(part 1 of 2)
# Autodesk Inventor assembly: woodhouseV1
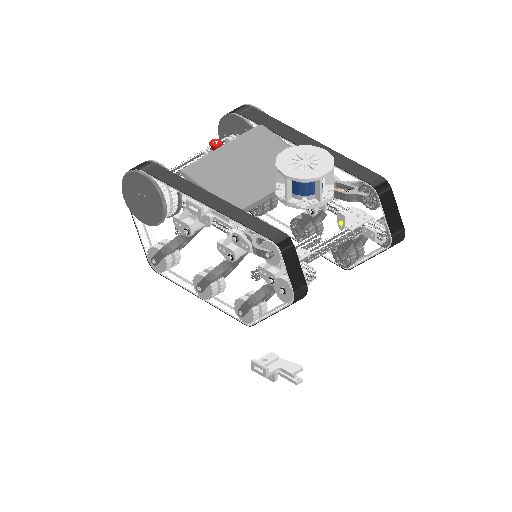
[picture p0: Inventor's stored thumbnail of the model, 512x512]
Saved by Autodesk Inventor 2025 (Build 290162000, 162)
## iProperties
Created: 2024-10-22
Part Number: woodhouseV1
Document SubType Name: Assembly
Designer: derm
Author: derm
## Documents named in this file (47)
- C:\Users\derm\Desktop\puppycat\woodhouseV1.iam
- C:\Users\derm\Desktop\puppycat\100MMshockUpper.ipt
- C:\Users\derm\Desktop\puppycat\100MMshockLower.ipt
- C:\Users\derm\Desktop\puppycat\swingarmBaseV2.ipt
- C:\Users\derm\Desktop\puppycat\6082rsBearing.ipt
- C:\Users\derm\Desktop\puppycat\92981A203_Alloy Steel Shoulder Screws\92981A203_Alloy Steel Shoulder Screws.ipt
- C:\Users\derm\Desktop\puppycat\swingarmV2.ipt
- C:\Users\derm\Desktop\puppycat\am-3298a 20 tooth Molded Tank Pulley Half Rev4\am-3298a 20 tooth Molded Tank Pulley Half Rev4.ipt
- C:\Users\derm\Desktop\puppycat\am3298_bearing_adapter.ipt
- C:\Users\derm\Desktop\puppycat\90237A130_High-Strength Steel Nylon-Insert Locknuts\90237A130_High-Strength Steel Nylon-Insert Locknuts.ipt
- C:\Users\derm\Desktop\puppycat\trackBase.ipt
- C:\Users\derm\Desktop\puppycat\moteur hoverboard\hoverboard_motor_assembly\hoverboard_motor_assembly.ipt
- C:\Users\derm\Desktop\puppycat\hoverboardPulleyAdapter.ipt
- C:\Users\derm\Desktop\puppycat\hoverboardMotorMount.ipt
- C:\Users\derm\Desktop\puppycat\idlerBaseV1.ipt
- C:\Users\derm\Desktop\puppycat\printedWheel.ipt
- C:\Users\derm\Desktop\puppycat\9002T445_Corrosion-Resistant Precision Compression Springs\9002T445_Corrosion-Resistant Precision Compression Springs.ipt
- C:\Users\derm\Desktop\puppycat\idlerV1.ipt
- C:\Users\derm\Desktop\puppycat\beltV2.ipt
- C:\Users\derm\Desktop\puppycat\springSpacerV1.ipt
- C:\Users\derm\Desktop\puppycat\swingarmBaseV4.ipt
- C:\Users\derm\Desktop\puppycat\swingarmBaseV4_mirror.ipt
- C:\Users\derm\Desktop\puppycat\swingarmV2_mirrored.ipt
- C:\Users\derm\Desktop\puppycat\91290A461_Alloy Steel Socket Head Screw\91290A461_Alloy Steel Socket Head Screw.ipt
- C:\Users\derm\Desktop\puppycat\94645A210_High-Strength Steel Nylon-Insert Locknut\94645A210_High-Strength Steel Nylon-Insert Locknut.ipt
- C:\Users\derm\Desktop\puppycat\91290A270_Alloy Steel Socket Head Screw\91290A270_Alloy Steel Socket Head Screw.ipt
- C:\Users\derm\Desktop\puppycat\horizontalStrut.ipt
- C:\Users\derm\Desktop\puppycat\4844N132_T-Slotted Framing Structural Bracket\4844N132_T-Slotted Framing Structural Bracket.ipt
- C:\Users\derm\Desktop\puppycat\4844N105_T-Slotted Framing Structural Bracket\4844N105_T-Slotted Framing Structural Bracket.ipt
- C:\Users\derm\Desktop\puppycat\lidarFOV.ipt
- C:\Users\derm\Desktop\puppycat\Motor driver ODRIVE V3.6\Motor driver ODRIVE V3.6.ipt
- C:\Users\derm\Desktop\puppycat\Zippy5000.ipt
- C:\Users\derm\Desktop\puppycat\50W 2Ohm Power Resistor\50W 2Ohm Power Resistor.ipt
- C:\Users\derm\Desktop\puppycat\odriveAndBatteryMountV1.ipt
- C:\Users\derm\Desktop\puppycat\E-STOP\E-STOP.ipt
- C:\Users\derm\Desktop\puppycat\estopMountV1.ipt
- C:\Users\derm\Desktop\puppycat\LAPTOP.iam
- C:\Users\derm\Desktop\puppycat\hoverboardHubCap.ipt
- C:\Users\derm\Desktop\puppycat\laptopClampBase.ipt
- C:\Users\derm\Desktop\puppycat\hoverboardInnerHubCap.ipt
- C:\Users\derm\Desktop\puppycat\dellLatitudeBase.ipt
- C:\Users\derm\Desktop\puppycat\dellLatitudeScreen.ipt
- C:\Users\derm\Desktop\puppycat\laptopClampScrew.ipt
- C:\Users\derm\Desktop\puppycat\laptopClampBaseFlipped.ipt
- C:\Users\derm\Desktop\puppycat\liarAssembly.iam
- C:\Users\derm\Desktop\puppycat\laptopClampBaseShort.ipt
- C:\Users\derm\Desktop\puppycat\12inStrut.ipt
## Components (214 placed, 46 different names)
1. 100MMshockUpper:1 — Mate:1, Angle:1, Mate:2, Mate:22, Mate:25, Mate:58, Mate:251, Mate:252, Mate:253
2. 100MMshockLower:1 — Mate:1, Angle:1, Mate:2, Mate:26, Mate:57
3. swingarmBaseV4:1 — Mate:3, Mate:4, Mate:19, Mate:22, Mate:25, Mate:27, Angle:2, Mate:33, Flush:3, Mate:39, Mate:40, Mate:41, Mate:253, Flush:10
4. 6082rsBearing:1 — Mate:3, Mate:4, Mate:16, Mate:17
5. 6082rsBearing:2 — Mate:18, Mate:19, Mate:21
6. 92981A203_Alloy Steel Shoulder Screws:1 — Mate:16, Mate:17, Mate:18, Mate:20, Mate:23
7. swingarmV2:1 — Mate:20, Mate:21, Mate:24, Mate:26, Mate:34, Mate:42, Flush:13
8. am-3298a 20 tooth Molded Tank Pulley Half Rev4:1
9. am-3298a 20 tooth Molded Tank Pulley Half Rev4:2 — Flush:2, Flush:4
10. 6082rsBearing:3 — Mate:34
11. 6082rsBearing:4
12. am3298_bearing_adapter:1
13. am3298_bearing_adapter:2
14. 90237A130_High-Strength Steel Nylon-Insert Locknuts:1 — Mate:23, Mate:24
15. trackBase:1 — Mate:27, Angle:2, Angle:3, Mate:32, Tangent:1, Mate:33, Flush:3, Mate:54, Mate:55, Mate:70, Mate:71, Mate:136, Mate:137, Mate:197, Mate:198, Mate:249, Mate:250, Flush:7, Flush:8, Mate:429, Mate:430, Flush:32, Mate:431, Flush:36, Flush:40, Mate:436, Mate:464, Mate:490, Mate:491, Mate:494, Flush:65, Flush:66
16. hoverboard_motor_assembly:1 — Angle:4, Flush:1, Mate:481, Mate:482, Mate:483, Mate:484, Mate:485
17. hoverboardPulleyAdapter:1 — Flush:2, Flush:5, Mate:468
18. hoverboardMotorMount:1 — Angle:3, Mate:32, Angle:4, Flush:1, Tangent:1
19. 6082rsBearing:5 — Mate:39
20. 6082rsBearing:6 — Mate:41
21. 92981A203_Alloy Steel Shoulder Screws:2 — Mate:40
22. 90237A130_High-Strength Steel Nylon-Insert Locknuts:2 — Mate:42
23. am-3298a 20 tooth Molded Tank Pulley Half Rev4:3
24. am-3298a 20 tooth Molded Tank Pulley Half Rev4:4 — Flush:4
25. 6082rsBearing:7
26. 6082rsBearing:8 — Mate:56
27. am3298_bearing_adapter:3
28. am3298_bearing_adapter:4
29. idlerBaseV1:1 — Mate:54, Mate:55, Mate:56, Flush:61
30. 9002T445_Corrosion-Resistant Precision Compression Springs:1 — Mate:57, Mate:58
31. idlerV1:1 — Mate:59, Mate:60, Mate:61, Mate:62, Flush:5
32. 6082rsBearing:9 — Mate:59, Mate:61
33. 6082rsBearing:10 — Mate:60, Mate:62, Mate:72
34. idlerBaseV1:3 — Mate:70, Mate:71, Mate:72
35. swingarmBaseV2:2 — Mate:136, Mate:137, Mate:144, Flush:21
36. 6082rsBearing:17
37. 6082rsBearing:18
38. 92981A203_Alloy Steel Shoulder Screws:4
39. swingarmV2:2 — Mate:138, Mate:139, Mate:145, Mate:146, Flush:23
40. am-3298a 20 tooth Molded Tank Pulley Half Rev4:5
41. am-3298a 20 tooth Molded Tank Pulley Half Rev4:6
42. 6082rsBearing:19
43. 6082rsBearing:20 — Mate:138, Mate:139
44. am3298_bearing_adapter:5
45. am3298_bearing_adapter:6
46. 90237A130_High-Strength Steel Nylon-Insert Locknuts:3
47. 6082rsBearing:21
48. 6082rsBearing:22
49. 92981A203_Alloy Steel Shoulder Screws:5
50. 90237A130_High-Strength Steel Nylon-Insert Locknuts:4
51. 100MMshockUpper:2 — Mate:144, Mate:146
52. 100MMshockLower:2 — Mate:145
53. 9002T445_Corrosion-Resistant Precision Compression Springs:2
54. 100MMshockUpper:3
55. 100MMshockLower:3
56. swingarmBaseV2:3 — Mate:197, Mate:198, Flush:22
57. 6082rsBearing:23
58. 6082rsBearing:24
59. 92981A203_Alloy Steel Shoulder Screws:6
60. swingarmV2:3 — Mate:196, Flush:24
61. am-3298a 20 tooth Molded Tank Pulley Half Rev4:7
62. am-3298a 20 tooth Molded Tank Pulley Half Rev4:8
63. 6082rsBearing:25
64. 6082rsBearing:26 — Mate:196
65. am3298_bearing_adapter:7
66. am3298_bearing_adapter:8
67. 90237A130_High-Strength Steel Nylon-Insert Locknuts:5
68. 6082rsBearing:27
69. 6082rsBearing:28
70. 92981A203_Alloy Steel Shoulder Screws:7
71. 90237A130_High-Strength Steel Nylon-Insert Locknuts:6
72. 9002T445_Corrosion-Resistant Precision Compression Springs:3
73. 100MMshockUpper:4
74. 100MMshockLower:4
75. swingarmBaseV2:4 — Mate:249, Mate:250, Flush:27
76. 6082rsBearing:29
77. 6082rsBearing:30
78. 92981A203_Alloy Steel Shoulder Screws:8
79. swingarmV2:4 — Mate:248, Flush:28
80. am-3298a 20 tooth Molded Tank Pulley Half Rev4:9
81. am-3298a 20 tooth Molded Tank Pulley Half Rev4:10
82. 6082rsBearing:31
83. 6082rsBearing:32 — Mate:248
84. am3298_bearing_adapter:9
85. am3298_bearing_adapter:10
86. 90237A130_High-Strength Steel Nylon-Insert Locknuts:7
87. 6082rsBearing:33
88. 6082rsBearing:34
89. 92981A203_Alloy Steel Shoulder Screws:9
90. 90237A130_High-Strength Steel Nylon-Insert Locknuts:8
91. 9002T445_Corrosion-Resistant Precision Compression Springs:4
92. beltV2:1 — Flush:29, Flush:30
93. springSpacerV1:1 — Mate:251, Mate:252
94. trackBase:2 — Flush:7, Flush:8, Mate:255, Mate:256, Mate:264, Mate:265, Mate:308, Flush:15, Flush:16, Mate:385, Mate:386, Mate:387, Mate:388, Mate:427, Mate:428, Mate:429, Mate:432, Flush:35, Flush:38, Mate:438, Mate:471, Flush:56
95. swingarmBaseV4_mirror:1 — Mate:264, Mate:265, Flush:10, Mate:266, Mate:267, Mate:268, Mate:270, Mate:274, Mate:275, Mate:291, Mate:293, Mate:294
96. swingarmV2_mirrored:1 — Mate:266, Mate:271, Mate:276, Mate:278, Mate:282, Mate:283, Mate:284, Angle:8, Flush:11, Mate:292, Flush:12, Flush:13, Mate:299, Mate:304
97. 6082rsBearing:35 — Mate:258, Mate:259, Mate:263
98. idlerBaseV1:4 — Mate:255, Mate:256, Mate:257, Mate:263, Flush:61
99. printedWheel:2 — Mate:257, Mate:259, Mate:260
100. 6082rsBearing:36 — Mate:258, Mate:260, Mate:261, Mate:262
101. 91290A461_Alloy Steel Socket Head Screw:1 — Mate:261, Mate:262
102. 6082rsBearing:37 — Mate:267, Mate:268, Mate:269, Mate:296, Mate:297
103. 6082rsBearing:38 — Mate:269, Mate:270, Mate:271
104. 6082rsBearing:39 — Mate:274, Mate:275, Mate:301, Mate:302
105. printedWheel:3 — Mate:276, Mate:277, Mate:279, Mate:280, Mate:281
106. 6082rsBearing:41 — Mate:280, Mate:281
107. 6082rsBearing:42 — Mate:277, Mate:278, Mate:279
108. 91290A461_Alloy Steel Socket Head Screw:2 — Mate:282, Mate:283
109. 94645A210_High-Strength Steel Nylon-Insert Locknut:1 — Mate:284, Angle:8, Flush:11
110. 100MMshockUpper:5 — Mate:291, Flush:12
111. 100MMshockLower:5 — Mate:292
112. 9002T445_Corrosion-Resistant Precision Compression Springs:5
113. springSpacerV1:2
114. 91290A270_Alloy Steel Socket Head Screw:1 — Mate:293, Mate:294
115. 92981A203_Alloy Steel Shoulder Screws:10 — Mate:296, Mate:297, Mate:298
116. 90237A130_High-Strength Steel Nylon-Insert Locknuts:9 — Mate:298, Mate:299
117. 92981A203_Alloy Steel Shoulder Screws:11 — Mate:301, Mate:302, Mate:303
118. 90237A130_High-Strength Steel Nylon-Insert Locknuts:10 — Mate:303, Mate:304
119. hoverboard_motor_assembly:2 — Mate:472, Mate:473, Mate:476, Mate:477, Mate:478
120. hoverboardPulleyAdapter:2 — Flush:31, Mate:469, Mate:470
121. hoverboardMotorMount:2 — Mate:308, Flush:15, Flush:16
122. swingarmBaseV4_mirror:2 — Mate:385, Mate:386, Flush:21
123. swingarmV2_mirrored:2 — Flush:23
124. 6082rsBearing:43
125. 6082rsBearing:44
126. 6082rsBearing:45
127. printedWheel:4
128. 6082rsBearing:47
129. 6082rsBearing:48
130. 91290A461_Alloy Steel Socket Head Screw:3
131. 94645A210_High-Strength Steel Nylon-Insert Locknut:2
132. 100MMshockUpper:6
133. 100MMshockLower:6
134. 9002T445_Corrosion-Resistant Precision Compression Springs:6
135. springSpacerV1:3
136. 91290A270_Alloy Steel Socket Head Screw:2
137. 92981A203_Alloy Steel Shoulder Screws:12
138. 90237A130_High-Strength Steel Nylon-Insert Locknuts:11
139. 92981A203_Alloy Steel Shoulder Screws:13
140. 90237A130_High-Strength Steel Nylon-Insert Locknuts:12
141. swingarmBaseV4_mirror:3 — Mate:387, Mate:388, Flush:22
142. swingarmV2_mirrored:3 — Flush:24
143. 6082rsBearing:49
144. 6082rsBearing:50
145. 6082rsBearing:51
146. printedWheel:5
147. 6082rsBearing:53
148. 6082rsBearing:54
149. 91290A461_Alloy Steel Socket Head Screw:4
150. 94645A210_High-Strength Steel Nylon-Insert Locknut:3
151. 100MMshockUpper:7
152. 100MMshockLower:7
153. 9002T445_Corrosion-Resistant Precision Compression Springs:7
154. springSpacerV1:4
155. 91290A270_Alloy Steel Socket Head Screw:3
156. 92981A203_Alloy Steel Shoulder Screws:14
157. 90237A130_High-Strength Steel Nylon-Insert Locknuts:13
158. 92981A203_Alloy Steel Shoulder Screws:15
159. 90237A130_High-Strength Steel Nylon-Insert Locknuts:14
160. swingarmBaseV4_mirror:4 — Mate:427, Mate:428, Flush:27
161. swingarmV2_mirrored:4 — Flush:28
162. 6082rsBearing:55
163. 6082rsBearing:56
164. 6082rsBearing:57
165. printedWheel:6
166. 6082rsBearing:59
167. 6082rsBearing:60
168. 91290A461_Alloy Steel Socket Head Screw:5
169. 94645A210_High-Strength Steel Nylon-Insert Locknut:4
170. 100MMshockUpper:8
171. 100MMshockLower:8
172. 9002T445_Corrosion-Resistant Precision Compression Springs:8
173. springSpacerV1:5
174. 91290A270_Alloy Steel Socket Head Screw:4
175. 92981A203_Alloy Steel Shoulder Screws:16
176. 90237A130_High-Strength Steel Nylon-Insert Locknuts:15
177. 92981A203_Alloy Steel Shoulder Screws:17
178. 90237A130_High-Strength Steel Nylon-Insert Locknuts:16
179. beltV2:2 — Flush:29, Flush:30, Flush:31
180. horizontalStrut:1 — Mate:430, Flush:32, Flush:33, Flush:34, Mate:433, Flush:37, Mate:466
181. horizontalStrut:2 — Flush:33, Mate:431, Mate:434, Flush:39, Mate:435, Flush:41, Mate:437, Flush:42, Mate:439, Mate:457, Mate:458, Mate:467, Flush:67
182. 4844N132_T-Slotted Framing Structural Bracket:1 — Mate:432, Flush:34, Flush:35
183. 4844N132_T-Slotted Framing Structural Bracket:2 — Mate:434, Flush:38, Flush:39
184. 4844N132_T-Slotted Framing Structural Bracket:3 — Mate:435, Flush:40, Flush:41
185. 4844N132_T-Slotted Framing Structural Bracket:4 — Mate:433, Flush:36, Flush:37
186. 4844N105_T-Slotted Framing Structural Bracket:1 — Mate:436, Mate:437, Flush:42, Flush:43
187. 4844N105_T-Slotted Framing Structural Bracket:2 — Mate:438, Mate:439, Flush:43
188. lidarFOV:1
189. Motor driver ODRIVE V3.6:1 — Mate:451, Mate:452, Mate:453
190. Zippy5000:1
191. 50W 2Ohm Power Resistor:1 — Mate:454, Mate:455, Mate:456
192. odriveAndBatteryMountV1:1 — Mate:451, Mate:452, Mate:453, Mate:454, Mate:455, Mate:456, Mate:457, Mate:458
193. E-STOP:1 — Mate:459, Mate:460, Mate:461
194. estopMountV1:1 — Mate:459, Mate:460, Mate:461, Mate:466, Mate:467
195. LAPTOP:1 [sub-assembly] — Mate:464
196. hoverboardHubCap:1 — Mate:468
197. hoverboardHubCap:2 — Mate:469, Mate:470
198. laptopClampBase:1 — Mate:471, Flush:56, Mate:488, Mate:489, Flush:62
199. hoverboardInnerHubCap:1 — Mate:472, Mate:473, Mate:474, Mate:475, Flush:57, Flush:58, Mate:476
200. hoverboardInnerHubCap:2 — Mate:474, Flush:57, Mate:478
201. hoverboardInnerHubCap:3 — Mate:475, Flush:58, Mate:477
202. hoverboardInnerHubCap:4 — Mate:481, Mate:482, Mate:483
203. hoverboardInnerHubCap:5 — Mate:484
204. hoverboardInnerHubCap:6 — Mate:485
205. dellLatitudeBase:1 — Mate:486, Mate:487
206. dellLatitudeScreen:1 — Mate:486, Mate:487
207. laptopClampScrew:1 — Mate:488, Mate:489
208. laptopClampBaseFlipped:1 — Mate:490, Mate:491, Flush:62, Mate:492, Mate:493
209. laptopClampScrew:2 — Mate:492, Mate:493
210. horizontalStrut:4 — Flush:63, Flush:64
211. horizontalStrut:5 — Flush:63, Flush:64, Flush:67
212. liarAssembly:1 [sub-assembly]
213. laptopClampBaseShort:1
214. 12inStrut:1 — Mate:494, Flush:65, Flush:66
## Relationships (480: Mate 410, Flush 53, Angle 16, Tangent 1)
- Mate:1: 100MMshockUpper:1 ↔ 100MMshockLower:1
- Angle:1 (0 deg): 100MMshockUpper:1 ↔ 100MMshockLower:1
- Mate:2 (102 mm): 100MMshockUpper:1 ↔ 100MMshockLower:1
- Mate:3: swingarmBaseV4:1 ↔ 6082rsBearing:1
- Mate:4: swingarmBaseV4:1 ↔ 6082rsBearing:1
- [Mate]: am-3298a 20 tooth Molded Tank Pulley Half Rev4:1 ↔ am-3298a 20 tooth Molded Tank Pulley Half Rev4:2
- [Mate]: am-3298a 20 tooth Molded Tank Pulley Half Rev4:1 ↔ am-3298a 20 tooth Molded Tank Pulley Half Rev4:2
- [Mate]: am-3298a 20 tooth Molded Tank Pulley Half Rev4:1 ↔ am-3298a 20 tooth Molded Tank Pulley Half Rev4:2
- [Mate]: 6082rsBearing:4 ↔ am3298_bearing_adapter:1
- [Mate]: am-3298a 20 tooth Molded Tank Pulley Half Rev4:2 ↔ am3298_bearing_adapter:1
- [Mate]: am-3298a 20 tooth Molded Tank Pulley Half Rev4:2 ↔ 6082rsBearing:4
- [Mate]: 6082rsBearing:4 ↔ am3298_bearing_adapter:1
- [Mate]: am-3298a 20 tooth Molded Tank Pulley Half Rev4:1 ↔ am3298_bearing_adapter:2
- [Mate]: am-3298a 20 tooth Molded Tank Pulley Half Rev4:1 ↔ am3298_bearing_adapter:2
- [Mate]: 6082rsBearing:3 ↔ am3298_bearing_adapter:2
- [Mate]: 6082rsBearing:3 ↔ am3298_bearing_adapter:2
- Mate:16: 6082rsBearing:1 ↔ 92981A203_Alloy Steel Shoulder Screws:1
- Mate:17: 6082rsBearing:1 ↔ 92981A203_Alloy Steel Shoulder Screws:1
- Mate:18: 6082rsBearing:2 ↔ 92981A203_Alloy Steel Shoulder Screws:1
- Mate:19: swingarmBaseV4:1 ↔ 6082rsBearing:2
- Mate:20: 92981A203_Alloy Steel Shoulder Screws:1 ↔ swingarmV2:1
- Mate:21 (0.5 mm): 6082rsBearing:2 ↔ swingarmV2:1
- Mate:22: 100MMshockUpper:1 ↔ swingarmBaseV4:1
- Mate:23: 92981A203_Alloy Steel Shoulder Screws:1 ↔ 90237A130_High-Strength Steel Nylon-Insert Locknuts:1
- Mate:24 (1 mm): swingarmV2:1 ↔ 90237A130_High-Strength Steel Nylon-Insert Locknuts:1
- Mate:25 (24 mm): 100MMshockUpper:1 ↔ swingarmBaseV4:1
- Mate:26: 100MMshockLower:1 ↔ swingarmV2:1
- Mate:27: swingarmBaseV4:1 ↔ trackBase:1
- Angle:2 (0 deg): swingarmBaseV4:1 ↔ trackBase:1
- [Mate]: hoverboard_motor_assembly:1 ↔ hoverboardPulleyAdapter:1
- [Mate]: hoverboard_motor_assembly:1 ↔ hoverboardPulleyAdapter:1
- [Mate]: hoverboard_motor_assembly:1 ↔ hoverboardMotorMount:1
- Angle:3 (0 deg): trackBase:1 ↔ hoverboardMotorMount:1
- Mate:32: trackBase:1 ↔ hoverboardMotorMount:1
- Angle:4 (0 deg): hoverboard_motor_assembly:1 ↔ hoverboardMotorMount:1
- Flush:1 (37 mm): hoverboard_motor_assembly:1 ↔ hoverboardMotorMount:1
- Tangent:1 (1 mm): trackBase:1 ↔ hoverboardMotorMount:1
- Flush:2: am-3298a 20 tooth Molded Tank Pulley Half Rev4:2 ↔ hoverboardPulleyAdapter:1
- Mate:33: swingarmBaseV4:1 ↔ trackBase:1
- Mate:34: swingarmV2:1 ↔ 6082rsBearing:3
- Flush:3 (-10 mm): swingarmBaseV4:1 ↔ trackBase:1
- [Mate]: 6082rsBearing:5 ↔ 92981A203_Alloy Steel Shoulder Screws:2
- [Mate]: 6082rsBearing:5 ↔ 92981A203_Alloy Steel Shoulder Screws:2
- [Mate]: 6082rsBearing:6 ↔ 92981A203_Alloy Steel Shoulder Screws:2
- [Mate]: 92981A203_Alloy Steel Shoulder Screws:2 ↔ 90237A130_High-Strength Steel Nylon-Insert Locknuts:2
- Mate:39: swingarmBaseV4:1 ↔ 6082rsBearing:5
- Mate:40: swingarmBaseV4:1 ↔ 92981A203_Alloy Steel Shoulder Screws:2
- Mate:41: swingarmBaseV4:1 ↔ 6082rsBearing:6
- Mate:42: swingarmV2:1 ↔ 90237A130_High-Strength Steel Nylon-Insert Locknuts:2
- [Mate]: am-3298a 20 tooth Molded Tank Pulley Half Rev4:3 ↔ am-3298a 20 tooth Molded Tank Pulley Half Rev4:4
- [Mate]: am-3298a 20 tooth Molded Tank Pulley Half Rev4:3 ↔ am-3298a 20 tooth Molded Tank Pulley Half Rev4:4
- [Mate]: am-3298a 20 tooth Molded Tank Pulley Half Rev4:3 ↔ am-3298a 20 tooth Molded Tank Pulley Half Rev4:4
- [Mate]: 6082rsBearing:8 ↔ am3298_bearing_adapter:3
- [Mate]: am-3298a 20 tooth Molded Tank Pulley Half Rev4:4 ↔ am3298_bearing_adapter:3
- [Mate]: am-3298a 20 tooth Molded Tank Pulley Half Rev4:4 ↔ 6082rsBearing:8
- [Mate]: 6082rsBearing:8 ↔ am3298_bearing_adapter:3
- [Mate]: am-3298a 20 tooth Molded Tank Pulley Half Rev4:3 ↔ am3298_bearing_adapter:4
- [Mate]: am-3298a 20 tooth Molded Tank Pulley Half Rev4:3 ↔ am3298_bearing_adapter:4
- [Mate]: 6082rsBearing:7 ↔ am3298_bearing_adapter:4
- [Mate]: 6082rsBearing:7 ↔ am3298_bearing_adapter:4
- Flush:4: am-3298a 20 tooth Molded Tank Pulley Half Rev4:2 ↔ am-3298a 20 tooth Molded Tank Pulley Half Rev4:4
- Mate:54: trackBase:1 ↔ idlerBaseV1:1
- Mate:55: trackBase:1 ↔ idlerBaseV1:1
- Mate:56: 6082rsBearing:8 ↔ idlerBaseV1:1
- Mate:57: 100MMshockLower:1 ↔ 9002T445_Corrosion-Resistant Precision Compression Springs:1
- Mate:58: 100MMshockUpper:1 ↔ 9002T445_Corrosion-Resistant Precision Compression Springs:1
- Mate:59: idlerV1:1 ↔ 6082rsBearing:9
- Mate:60: idlerV1:1 ↔ 6082rsBearing:10
- Mate:61: idlerV1:1 ↔ 6082rsBearing:9
- Mate:62: idlerV1:1 ↔ 6082rsBearing:10
- Flush:5: hoverboardPulleyAdapter:1 ↔ idlerV1:1
- Mate:70: trackBase:1 ↔ idlerBaseV1:3
- Mate:71: trackBase:1 ↔ idlerBaseV1:3
- Mate:72: 6082rsBearing:10 ↔ idlerBaseV1:3
- [Mate]: swingarmBaseV2:2 ↔ 6082rsBearing:17
- [Mate]: swingarmBaseV2:2 ↔ 6082rsBearing:17
- [Mate]: am-3298a 20 tooth Molded Tank Pulley Half Rev4:5 ↔ am-3298a 20 tooth Molded Tank Pulley Half Rev4:6
- [Mate]: am-3298a 20 tooth Molded Tank Pulley Half Rev4:5 ↔ am-3298a 20 tooth Molded Tank Pulley Half Rev4:6
- [Mate]: am-3298a 20 tooth Molded Tank Pulley Half Rev4:5 ↔ am-3298a 20 tooth Molded Tank Pulley Half Rev4:6
- [Mate]: 6082rsBearing:20 ↔ am3298_bearing_adapter:5
- [Mate]: am-3298a 20 tooth Molded Tank Pulley Half Rev4:6 ↔ am3298_bearing_adapter:5
- [Mate]: am-3298a 20 tooth Molded Tank Pulley Half Rev4:6 ↔ 6082rsBearing:20
- [Mate]: 6082rsBearing:20 ↔ am3298_bearing_adapter:5
- [Mate]: am-3298a 20 tooth Molded Tank Pulley Half Rev4:5 ↔ am3298_bearing_adapter:6
- [Mate]: am-3298a 20 tooth Molded Tank Pulley Half Rev4:5 ↔ am3298_bearing_adapter:6
- [Mate]: 6082rsBearing:19 ↔ am3298_bearing_adapter:6
- [Mate]: 6082rsBearing:19 ↔ am3298_bearing_adapter:6
- [Mate]: 6082rsBearing:17 ↔ 92981A203_Alloy Steel Shoulder Screws:4
- [Mate]: 6082rsBearing:17 ↔ 92981A203_Alloy Steel Shoulder Screws:4
- [Mate]: 6082rsBearing:18 ↔ 92981A203_Alloy Steel Shoulder Screws:4
- [Mate]: swingarmBaseV2:2 ↔ 6082rsBearing:18
- [Mate]: 92981A203_Alloy Steel Shoulder Screws:4 ↔ swingarmV2:2
- [Mate] (0.5 mm): 6082rsBearing:18 ↔ swingarmV2:2
- [Mate]: 92981A203_Alloy Steel Shoulder Screws:4 ↔ 90237A130_High-Strength Steel Nylon-Insert Locknuts:3
- [Mate] (1 mm): swingarmV2:2 ↔ 90237A130_High-Strength Steel Nylon-Insert Locknuts:3
- [Mate]: swingarmV2:2 ↔ 6082rsBearing:19
- [Mate]: 6082rsBearing:21 ↔ 92981A203_Alloy Steel Shoulder Screws:5
- [Mate]: 6082rsBearing:21 ↔ 92981A203_Alloy Steel Shoulder Screws:5
- [Mate]: 6082rsBearing:22 ↔ 92981A203_Alloy Steel Shoulder Screws:5
- [Mate]: 92981A203_Alloy Steel Shoulder Screws:5 ↔ 90237A130_High-Strength Steel Nylon-Insert Locknuts:4
- [Mate]: swingarmBaseV2:2 ↔ 6082rsBearing:21
- [Mate]: swingarmBaseV2:2 ↔ 92981A203_Alloy Steel Shoulder Screws:5
- [Mate]: swingarmBaseV2:2 ↔ 6082rsBearing:22
- [Mate]: swingarmV2:2 ↔ 90237A130_High-Strength Steel Nylon-Insert Locknuts:4
- Mate:136: trackBase:1 ↔ swingarmBaseV2:2
- Mate:137: trackBase:1 ↔ swingarmBaseV2:2
- Mate:138: swingarmV2:2 ↔ 6082rsBearing:20
- Mate:139 (1 mm): swingarmV2:2 ↔ 6082rsBearing:20
- [Mate]: 100MMshockUpper:2 ↔ 100MMshockLower:2
- [Angle] (0 deg): 100MMshockUpper:2 ↔ 100MMshockLower:2
- [Mate] (102 mm): 100MMshockUpper:2 ↔ 100MMshockLower:2
- [Mate]: 100MMshockLower:2 ↔ 9002T445_Corrosion-Resistant Precision Compression Springs:2
- [Mate]: 100MMshockUpper:2 ↔ 9002T445_Corrosion-Resistant Precision Compression Springs:2
- Mate:144: swingarmBaseV2:2 ↔ 100MMshockUpper:2
- Mate:145: swingarmV2:2 ↔ 100MMshockLower:2
- Mate:146: swingarmV2:2 ↔ 100MMshockUpper:2
- [Mate]: 100MMshockUpper:3 ↔ 100MMshockLower:3
- [Angle] (0 deg): 100MMshockUpper:3 ↔ 100MMshockLower:3
- [Mate] (102 mm): 100MMshockUpper:3 ↔ 100MMshockLower:3
- [Mate]: swingarmBaseV2:3 ↔ 6082rsBearing:23
- [Mate]: swingarmBaseV2:3 ↔ 6082rsBearing:23
- [Mate]: am-3298a 20 tooth Molded Tank Pulley Half Rev4:7 ↔ am-3298a 20 tooth Molded Tank Pulley Half Rev4:8
- [Mate]: am-3298a 20 tooth Molded Tank Pulley Half Rev4:7 ↔ am-3298a 20 tooth Molded Tank Pulley Half Rev4:8
- [Mate]: am-3298a 20 tooth Molded Tank Pulley Half Rev4:7 ↔ am-3298a 20 tooth Molded Tank Pulley Half Rev4:8
- [Mate]: 6082rsBearing:26 ↔ am3298_bearing_adapter:7
- [Mate]: am-3298a 20 tooth Molded Tank Pulley Half Rev4:8 ↔ am3298_bearing_adapter:7
- [Mate]: am-3298a 20 tooth Molded Tank Pulley Half Rev4:8 ↔ 6082rsBearing:26
- [Mate]: 6082rsBearing:26 ↔ am3298_bearing_adapter:7
- [Mate]: am-3298a 20 tooth Molded Tank Pulley Half Rev4:7 ↔ am3298_bearing_adapter:8
- [Mate]: am-3298a 20 tooth Molded Tank Pulley Half Rev4:7 ↔ am3298_bearing_adapter:8
- [Mate]: 6082rsBearing:25 ↔ am3298_bearing_adapter:8
- [Mate]: 6082rsBearing:25 ↔ am3298_bearing_adapter:8
- [Mate]: 6082rsBearing:23 ↔ 92981A203_Alloy Steel Shoulder Screws:6
- [Mate]: 6082rsBearing:23 ↔ 92981A203_Alloy Steel Shoulder Screws:6
- [Mate]: 6082rsBearing:24 ↔ 92981A203_Alloy Steel Shoulder Screws:6
- [Mate]: swingarmBaseV2:3 ↔ 6082rsBearing:24
- [Mate]: 92981A203_Alloy Steel Shoulder Screws:6 ↔ swingarmV2:3
- [Mate] (0.5 mm): 6082rsBearing:24 ↔ swingarmV2:3
- [Mate]: 100MMshockUpper:3 ↔ swingarmBaseV2:3
- [Mate]: 92981A203_Alloy Steel Shoulder Screws:6 ↔ 90237A130_High-Strength Steel Nylon-Insert Locknuts:5
- [Mate] (1 mm): swingarmV2:3 ↔ 90237A130_High-Strength Steel Nylon-Insert Locknuts:5
- [Mate] (24 mm): 100MMshockUpper:3 ↔ swingarmBaseV2:3
- [Mate]: 100MMshockLower:3 ↔ swingarmV2:3
- [Mate]: swingarmV2:3 ↔ 6082rsBearing:25
- [Mate]: 6082rsBearing:27 ↔ 92981A203_Alloy Steel Shoulder Screws:7
- [Mate]: 6082rsBearing:27 ↔ 92981A203_Alloy Steel Shoulder Screws:7
- [Mate]: 6082rsBearing:28 ↔ 92981A203_Alloy Steel Shoulder Screws:7
- [Mate]: 92981A203_Alloy Steel Shoulder Screws:7 ↔ 90237A130_High-Strength Steel Nylon-Insert Locknuts:6
- [Mate]: swingarmBaseV2:3 ↔ 6082rsBearing:27
- [Mate]: swingarmBaseV2:3 ↔ 92981A203_Alloy Steel Shoulder Screws:7
- [Mate]: swingarmBaseV2:3 ↔ 6082rsBearing:28
- [Mate]: swingarmV2:3 ↔ 90237A130_High-Strength Steel Nylon-Insert Locknuts:6
- [Mate]: 100MMshockLower:3 ↔ 9002T445_Corrosion-Resistant Precision Compression Springs:3
- [Mate]: 100MMshockUpper:3 ↔ 9002T445_Corrosion-Resistant Precision Compression Springs:3
- Mate:196 (1 mm): swingarmV2:3 ↔ 6082rsBearing:26
- Mate:197: trackBase:1 ↔ swingarmBaseV2:3
- Mate:198: trackBase:1 ↔ swingarmBaseV2:3
- [Mate]: 100MMshockUpper:4 ↔ 100MMshockLower:4
- [Angle] (0 deg): 100MMshockUpper:4 ↔ 100MMshockLower:4
- [Mate] (102 mm): 100MMshockUpper:4 ↔ 100MMshockLower:4
- [Mate]: swingarmBaseV2:4 ↔ 6082rsBearing:29
- [Mate]: swingarmBaseV2:4 ↔ 6082rsBearing:29
- [Mate]: am-3298a 20 tooth Molded Tank Pulley Half Rev4:9 ↔ am-3298a 20 tooth Molded Tank Pulley Half Rev4:10
- [Mate]: am-3298a 20 tooth Molded Tank Pulley Half Rev4:9 ↔ am-3298a 20 tooth Molded Tank Pulley Half Rev4:10
- [Mate]: am-3298a 20 tooth Molded Tank Pulley Half Rev4:9 ↔ am-3298a 20 tooth Molded Tank Pulley Half Rev4:10
- [Mate]: 6082rsBearing:32 ↔ am3298_bearing_adapter:9
- [Mate]: am-3298a 20 tooth Molded Tank Pulley Half Rev4:10 ↔ am3298_bearing_adapter:9
- [Mate]: am-3298a 20 tooth Molded Tank Pulley Half Rev4:10 ↔ 6082rsBearing:32
- [Mate]: 6082rsBearing:32 ↔ am3298_bearing_adapter:9
- [Mate]: am-3298a 20 tooth Molded Tank Pulley Half Rev4:9 ↔ am3298_bearing_adapter:10
- [Mate]: am-3298a 20 tooth Molded Tank Pulley Half Rev4:9 ↔ am3298_bearing_adapter:10
- [Mate]: 6082rsBearing:31 ↔ am3298_bearing_adapter:10
- [Mate]: 6082rsBearing:31 ↔ am3298_bearing_adapter:10
- [Mate]: 6082rsBearing:29 ↔ 92981A203_Alloy Steel Shoulder Screws:8
- [Mate]: 6082rsBearing:29 ↔ 92981A203_Alloy Steel Shoulder Screws:8
- [Mate]: 6082rsBearing:30 ↔ 92981A203_Alloy Steel Shoulder Screws:8
- [Mate]: swingarmBaseV2:4 ↔ 6082rsBearing:30
- [Mate]: 92981A203_Alloy Steel Shoulder Screws:8 ↔ swingarmV2:4
- [Mate] (0.5 mm): 6082rsBearing:30 ↔ swingarmV2:4
- [Mate]: 100MMshockUpper:4 ↔ swingarmBaseV2:4
- [Mate]: 92981A203_Alloy Steel Shoulder Screws:8 ↔ 90237A130_High-Strength Steel Nylon-Insert Locknuts:7
- [Mate] (1 mm): swingarmV2:4 ↔ 90237A130_High-Strength Steel Nylon-Insert Locknuts:7
- [Mate] (24 mm): 100MMshockUpper:4 ↔ swingarmBaseV2:4
- [Mate]: 100MMshockLower:4 ↔ swingarmV2:4
- [Mate]: swingarmV2:4 ↔ 6082rsBearing:31
- [Mate]: 6082rsBearing:33 ↔ 92981A203_Alloy Steel Shoulder Screws:9
- [Mate]: 6082rsBearing:33 ↔ 92981A203_Alloy Steel Shoulder Screws:9
- [Mate]: 6082rsBearing:34 ↔ 92981A203_Alloy Steel Shoulder Screws:9
- [Mate]: 92981A203_Alloy Steel Shoulder Screws:9 ↔ 90237A130_High-Strength Steel Nylon-Insert Locknuts:8
- [Mate]: swingarmBaseV2:4 ↔ 6082rsBearing:33
- [Mate]: swingarmBaseV2:4 ↔ 92981A203_Alloy Steel Shoulder Screws:9
- [Mate]: swingarmBaseV2:4 ↔ 6082rsBearing:34
- [Mate]: swingarmV2:4 ↔ 90237A130_High-Strength Steel Nylon-Insert Locknuts:8
- [Mate]: 100MMshockLower:4 ↔ 9002T445_Corrosion-Resistant Precision Compression Springs:4
- [Mate]: 100MMshockUpper:4 ↔ 9002T445_Corrosion-Resistant Precision Compression Springs:4
- Mate:248 (1 mm): swingarmV2:4 ↔ 6082rsBearing:32
- Mate:249: trackBase:1 ↔ swingarmBaseV2:4
- Mate:250: trackBase:1 ↔ swingarmBaseV2:4
- Mate:251: 100MMshockUpper:1 ↔ springSpacerV1:1
- Mate:252: 100MMshockUpper:1 ↔ springSpacerV1:1
- Mate:253: 100MMshockUpper:1 ↔ swingarmBaseV4:1
- Flush:7: trackBase:1 ↔ trackBase:2
- Flush:8: trackBase:1 ↔ trackBase:2
- [Mate]: 6082rsBearing:35 ↔ idlerBaseV1:4
- Mate:255: trackBase:2 ↔ idlerBaseV1:4
- Mate:256: trackBase:2 ↔ idlerBaseV1:4
- Mate:257: idlerBaseV1:4 ↔ printedWheel:2
- Mate:258: 6082rsBearing:35 ↔ 6082rsBearing:36
- Mate:259: 6082rsBearing:35 ↔ printedWheel:2
- Mate:260: printedWheel:2 ↔ 6082rsBearing:36
- Mate:261: 6082rsBearing:36 ↔ 91290A461_Alloy Steel Socket Head Screw:1
- Mate:262: 6082rsBearing:36 ↔ 91290A461_Alloy Steel Socket Head Screw:1
- Mate:263 (1 mm): 6082rsBearing:35 ↔ idlerBaseV1:4
- Mate:264: trackBase:2 ↔ swingarmBaseV4_mirror:1
- Mate:265: trackBase:2 ↔ swingarmBaseV4_mirror:1
- Flush:10: swingarmBaseV4:1 ↔ swingarmBaseV4_mirror:1
- Mate:266: swingarmBaseV4_mirror:1 ↔ swingarmV2_mirrored:1
- Mate:267: swingarmBaseV4_mirror:1 ↔ 6082rsBearing:37
- Mate:268: swingarmBaseV4_mirror:1 ↔ 6082rsBearing:37
- Mate:269: 6082rsBearing:37 ↔ 6082rsBearing:38
- Mate:270: swingarmBaseV4_mirror:1 ↔ 6082rsBearing:38
- Mate:271 (1 mm): swingarmV2_mirrored:1 ↔ 6082rsBearing:38
- Mate:274: swingarmBaseV4_mirror:1 ↔ 6082rsBearing:39
- Mate:275: swingarmBaseV4_mirror:1 ↔ 6082rsBearing:39
- Mate:276: swingarmV2_mirrored:1 ↔ printedWheel:3
- Mate:277: printedWheel:3 ↔ 6082rsBearing:42
- Mate:278 (0.5 mm): swingarmV2_mirrored:1 ↔ 6082rsBearing:42
- Mate:279: printedWheel:3 ↔ 6082rsBearing:42
- Mate:280: printedWheel:3 ↔ 6082rsBearing:41
- Mate:281: printedWheel:3 ↔ 6082rsBearing:41
- Mate:282: swingarmV2_mirrored:1 ↔ 91290A461_Alloy Steel Socket Head Screw:2
- Mate:283: swingarmV2_mirrored:1 ↔ 91290A461_Alloy Steel Socket Head Screw:2
- Mate:284: swingarmV2_mirrored:1 ↔ 94645A210_High-Strength Steel Nylon-Insert Locknut:1
- Angle:8 (0 deg): swingarmV2_mirrored:1 ↔ 94645A210_High-Strength Steel Nylon-Insert Locknut:1
- Flush:11: swingarmV2_mirrored:1 ↔ 94645A210_High-Strength Steel Nylon-Insert Locknut:1
- [Mate]: 100MMshockUpper:5 ↔ 100MMshockLower:5
- [Angle] (0 deg): 100MMshockUpper:5 ↔ 100MMshockLower:5
- [Mate] (102 mm): 100MMshockUpper:5 ↔ 100MMshockLower:5
- [Mate]: 100MMshockLower:5 ↔ 9002T445_Corrosion-Resistant Precision Compression Springs:5
- [Mate]: 100MMshockUpper:5 ↔ 9002T445_Corrosion-Resistant Precision Compression Springs:5
- [Mate]: 100MMshockUpper:5 ↔ springSpacerV1:2
- [Mate]: 100MMshockUpper:5 ↔ springSpacerV1:2
- Mate:291: swingarmBaseV4_mirror:1 ↔ 100MMshockUpper:5
- Mate:292: swingarmV2_mirrored:1 ↔ 100MMshockLower:5
- Flush:12 (-2 mm): swingarmV2_mirrored:1 ↔ 100MMshockUpper:5
- Mate:293: swingarmBaseV4_mirror:1 ↔ 91290A270_Alloy Steel Socket Head Screw:1
- Mate:294: swingarmBaseV4_mirror:1 ↔ 91290A270_Alloy Steel Socket Head Screw:1
- Flush:13: swingarmV2:1 ↔ swingarmV2_mirrored:1
- [Mate]: 92981A203_Alloy Steel Shoulder Screws:10 ↔ 90237A130_High-Strength Steel Nylon-Insert Locknuts:9
- Mate:296: 6082rsBearing:37 ↔ 92981A203_Alloy Steel Shoulder Screws:10
- Mate:297: 6082rsBearing:37 ↔ 92981A203_Alloy Steel Shoulder Screws:10
- Mate:298: 92981A203_Alloy Steel Shoulder Screws:10 ↔ 90237A130_High-Strength Steel Nylon-Insert Locknuts:9
- Mate:299: swingarmV2_mirrored:1 ↔ 90237A130_High-Strength Steel Nylon-Insert Locknuts:9
- [Mate]: 92981A203_Alloy Steel Shoulder Screws:11 ↔ 90237A130_High-Strength Steel Nylon-Insert Locknuts:10
- Mate:301: 6082rsBearing:39 ↔ 92981A203_Alloy Steel Shoulder Screws:11
- Mate:302: 6082rsBearing:39 ↔ 92981A203_Alloy Steel Shoulder Screws:11
- Mate:303: 92981A203_Alloy Steel Shoulder Screws:11 ↔ 90237A130_High-Strength Steel Nylon-Insert Locknuts:10
- Mate:304: swingarmV2_mirrored:1 ↔ 90237A130_High-Strength Steel Nylon-Insert Locknuts:10
- [Mate]: hoverboard_motor_assembly:2 ↔ hoverboardPulleyAdapter:2
- [Mate]: hoverboard_motor_assembly:2 ↔ hoverboardPulleyAdapter:2
- [Mate]: hoverboard_motor_assembly:2 ↔ hoverboardMotorMount:2
- [Angle] (0 deg): hoverboard_motor_assembly:2 ↔ hoverboardMotorMount:2
- [Flush] (37 mm): hoverboard_motor_assembly:2 ↔ hoverboardMotorMount:2
- Mate:308: trackBase:2 ↔ hoverboardMotorMount:2
- Flush:15: trackBase:2 ↔ hoverboardMotorMount:2
- Flush:16: trackBase:2 ↔ hoverboardMotorMount:2
- [Mate]: swingarmBaseV4_mirror:2 ↔ swingarmV2_mirrored:2
- [Mate]: swingarmBaseV4_mirror:2 ↔ 6082rsBearing:43
- [Mate]: swingarmBaseV4_mirror:2 ↔ 6082rsBearing:43
- [Mate]: 6082rsBearing:43 ↔ 6082rsBearing:44
- [Mate]: swingarmBaseV4_mirror:2 ↔ 6082rsBearing:44
- [Mate] (1 mm): swingarmV2_mirrored:2 ↔ 6082rsBearing:44
- [Mate]: swingarmBaseV4_mirror:2 ↔ 6082rsBearing:45
- [Mate]: swingarmBaseV4_mirror:2 ↔ 6082rsBearing:45
- [Mate]: swingarmV2_mirrored:2 ↔ printedWheel:4
- [Mate]: printedWheel:4 ↔ 6082rsBearing:48
- [Mate] (0.5 mm): swingarmV2_mirrored:2 ↔ 6082rsBearing:48
- [Mate]: printedWheel:4 ↔ 6082rsBearing:48
- [Mate]: printedWheel:4 ↔ 6082rsBearing:47
- [Mate]: printedWheel:4 ↔ 6082rsBearing:47
- [Mate]: swingarmV2_mirrored:2 ↔ 91290A461_Alloy Steel Socket Head Screw:3
- [Mate]: swingarmV2_mirrored:2 ↔ 91290A461_Alloy Steel Socket Head Screw:3
- [Mate]: swingarmV2_mirrored:2 ↔ 94645A210_High-Strength Steel Nylon-Insert Locknut:2
- [Angle] (0 deg): swingarmV2_mirrored:2 ↔ 94645A210_High-Strength Steel Nylon-Insert Locknut:2
- [Flush]: swingarmV2_mirrored:2 ↔ 94645A210_High-Strength Steel Nylon-Insert Locknut:2
- [Mate]: 100MMshockUpper:6 ↔ 100MMshockLower:6
- [Angle] (0 deg): 100MMshockUpper:6 ↔ 100MMshockLower:6
- [Mate] (102 mm): 100MMshockUpper:6 ↔ 100MMshockLower:6
- [Mate]: 100MMshockLower:6 ↔ 9002T445_Corrosion-Resistant Precision Compression Springs:6
- [Mate]: 100MMshockUpper:6 ↔ 9002T445_Corrosion-Resistant Precision Compression Springs:6
- [Mate]: 100MMshockUpper:6 ↔ springSpacerV1:3
- [Mate]: 100MMshockUpper:6 ↔ springSpacerV1:3
- [Mate]: swingarmBaseV4_mirror:2 ↔ 100MMshockUpper:6
- [Mate]: swingarmV2_mirrored:2 ↔ 100MMshockLower:6
- [Flush] (-2 mm): swingarmV2_mirrored:2 ↔ 100MMshockUpper:6
- [Mate]: swingarmBaseV4_mirror:2 ↔ 91290A270_Alloy Steel Socket Head Screw:2
- [Mate]: swingarmBaseV4_mirror:2 ↔ 91290A270_Alloy Steel Socket Head Screw:2
- [Mate]: 92981A203_Alloy Steel Shoulder Screws:12 ↔ 90237A130_High-Strength Steel Nylon-Insert Locknuts:11
- [Mate]: 6082rsBearing:43 ↔ 92981A203_Alloy Steel Shoulder Screws:12
- [Mate]: 6082rsBearing:43 ↔ 92981A203_Alloy Steel Shoulder Screws:12
- [Mate]: 92981A203_Alloy Steel Shoulder Screws:12 ↔ 90237A130_High-Strength Steel Nylon-Insert Locknuts:11
- [Mate]: swingarmV2_mirrored:2 ↔ 90237A130_High-Strength Steel Nylon-Insert Locknuts:11
- [Mate]: 92981A203_Alloy Steel Shoulder Screws:13 ↔ 90237A130_High-Strength Steel Nylon-Insert Locknuts:12
- [Mate]: 6082rsBearing:45 ↔ 92981A203_Alloy Steel Shoulder Screws:13
- [Mate]: 6082rsBearing:45 ↔ 92981A203_Alloy Steel Shoulder Screws:13
- [Mate]: 92981A203_Alloy Steel Shoulder Screws:13 ↔ 90237A130_High-Strength Steel Nylon-Insert Locknuts:12
- [Mate]: swingarmV2_mirrored:2 ↔ 90237A130_High-Strength Steel Nylon-Insert Locknuts:12
- [Mate]: swingarmBaseV4_mirror:3 ↔ swingarmV2_mirrored:3
- [Mate]: swingarmBaseV4_mirror:3 ↔ 6082rsBearing:49
- [Mate]: swingarmBaseV4_mirror:3 ↔ 6082rsBearing:49
- [Mate]: 6082rsBearing:49 ↔ 6082rsBearing:50
- [Mate]: swingarmBaseV4_mirror:3 ↔ 6082rsBearing:50
- [Mate] (1 mm): swingarmV2_mirrored:3 ↔ 6082rsBearing:50
- [Mate]: swingarmBaseV4_mirror:3 ↔ 6082rsBearing:51
- [Mate]: swingarmBaseV4_mirror:3 ↔ 6082rsBearing:51
- [Mate]: swingarmV2_mirrored:3 ↔ printedWheel:5
- [Mate]: printedWheel:5 ↔ 6082rsBearing:54
- [Mate] (0.5 mm): swingarmV2_mirrored:3 ↔ 6082rsBearing:54
- [Mate]: printedWheel:5 ↔ 6082rsBearing:54
- [Mate]: printedWheel:5 ↔ 6082rsBearing:53
- [Mate]: printedWheel:5 ↔ 6082rsBearing:53
- [Mate]: swingarmV2_mirrored:3 ↔ 91290A461_Alloy Steel Socket Head Screw:4
- [Mate]: swingarmV2_mirrored:3 ↔ 91290A461_Alloy Steel Socket Head Screw:4
- [Mate]: swingarmV2_mirrored:3 ↔ 94645A210_High-Strength Steel Nylon-Insert Locknut:3
- [Angle] (0 deg): swingarmV2_mirrored:3 ↔ 94645A210_High-Strength Steel Nylon-Insert Locknut:3
- [Flush]: swingarmV2_mirrored:3 ↔ 94645A210_High-Strength Steel Nylon-Insert Locknut:3
- [Mate]: 100MMshockUpper:7 ↔ 100MMshockLower:7
- [Angle] (0 deg): 100MMshockUpper:7 ↔ 100MMshockLower:7
- [Mate] (102 mm): 100MMshockUpper:7 ↔ 100MMshockLower:7
- [Mate]: 100MMshockLower:7 ↔ 9002T445_Corrosion-Resistant Precision Compression Springs:7
- [Mate]: 100MMshockUpper:7 ↔ 9002T445_Corrosion-Resistant Precision Compression Springs:7
- [Mate]: 100MMshockUpper:7 ↔ springSpacerV1:4
- [Mate]: 100MMshockUpper:7 ↔ springSpacerV1:4
- [Mate]: swingarmBaseV4_mirror:3 ↔ 100MMshockUpper:7
- [Mate]: swingarmV2_mirrored:3 ↔ 100MMshockLower:7
- [Flush] (-2 mm): swingarmV2_mirrored:3 ↔ 100MMshockUpper:7
- [Mate]: swingarmBaseV4_mirror:3 ↔ 91290A270_Alloy Steel Socket Head Screw:3
- [Mate]: swingarmBaseV4_mirror:3 ↔ 91290A270_Alloy Steel Socket Head Screw:3
- [Mate]: 92981A203_Alloy Steel Shoulder Screws:14 ↔ 90237A130_High-Strength Steel Nylon-Insert Locknuts:13
- [Mate]: 6082rsBearing:49 ↔ 92981A203_Alloy Steel Shoulder Screws:14
- [Mate]: 6082rsBearing:49 ↔ 92981A203_Alloy Steel Shoulder Screws:14
- [Mate]: 92981A203_Alloy Steel Shoulder Screws:14 ↔ 90237A130_High-Strength Steel Nylon-Insert Locknuts:13
- [Mate]: swingarmV2_mirrored:3 ↔ 90237A130_High-Strength Steel Nylon-Insert Locknuts:13
- [Mate]: 92981A203_Alloy Steel Shoulder Screws:15 ↔ 90237A130_High-Strength Steel Nylon-Insert Locknuts:14
- [Mate]: 6082rsBearing:51 ↔ 92981A203_Alloy Steel Shoulder Screws:15
- [Mate]: 6082rsBearing:51 ↔ 92981A203_Alloy Steel Shoulder Screws:15
- [Mate]: 92981A203_Alloy Steel Shoulder Screws:15 ↔ 90237A130_High-Strength Steel Nylon-Insert Locknuts:14
- [Mate]: swingarmV2_mirrored:3 ↔ 90237A130_High-Strength Steel Nylon-Insert Locknuts:14
- Mate:385: trackBase:2 ↔ swingarmBaseV4_mirror:2
- Mate:386: trackBase:2 ↔ swingarmBaseV4_mirror:2
- Flush:21: swingarmBaseV2:2 ↔ swingarmBaseV4_mirror:2
- Mate:387: trackBase:2 ↔ swingarmBaseV4_mirror:3
- Mate:388: trackBase:2 ↔ swingarmBaseV4_mirror:3
- Flush:22: swingarmBaseV2:3 ↔ swingarmBaseV4_mirror:3
- Flush:23: swingarmV2:2 ↔ swingarmV2_mirrored:2
- Flush:24: swingarmV2:3 ↔ swingarmV2_mirrored:3
- [Mate]: swingarmBaseV4_mirror:4 ↔ swingarmV2_mirrored:4
- [Mate]: swingarmBaseV4_mirror:4 ↔ 6082rsBearing:55
- [Mate]: swingarmBaseV4_mirror:4 ↔ 6082rsBearing:55
- [Mate]: 6082rsBearing:55 ↔ 6082rsBearing:56
- [Mate]: swingarmBaseV4_mirror:4 ↔ 6082rsBearing:56
- [Mate] (1 mm): swingarmV2_mirrored:4 ↔ 6082rsBearing:56
- [Mate]: swingarmBaseV4_mirror:4 ↔ 6082rsBearing:57
- [Mate]: swingarmBaseV4_mirror:4 ↔ 6082rsBearing:57
- [Mate]: swingarmV2_mirrored:4 ↔ printedWheel:6
- [Mate]: printedWheel:6 ↔ 6082rsBearing:60
- [Mate] (0.5 mm): swingarmV2_mirrored:4 ↔ 6082rsBearing:60
- [Mate]: printedWheel:6 ↔ 6082rsBearing:60
- [Mate]: printedWheel:6 ↔ 6082rsBearing:59
- [Mate]: printedWheel:6 ↔ 6082rsBearing:59
- [Mate]: swingarmV2_mirrored:4 ↔ 91290A461_Alloy Steel Socket Head Screw:5
- [Mate]: swingarmV2_mirrored:4 ↔ 91290A461_Alloy Steel Socket Head Screw:5
- [Mate]: swingarmV2_mirrored:4 ↔ 94645A210_High-Strength Steel Nylon-Insert Locknut:4
- [Angle] (0 deg): swingarmV2_mirrored:4 ↔ 94645A210_High-Strength Steel Nylon-Insert Locknut:4
- [Flush]: swingarmV2_mirrored:4 ↔ 94645A210_High-Strength Steel Nylon-Insert Locknut:4
- [Mate]: 100MMshockUpper:8 ↔ 100MMshockLower:8
- [Angle] (0 deg): 100MMshockUpper:8 ↔ 100MMshockLower:8
- [Mate] (102 mm): 100MMshockUpper:8 ↔ 100MMshockLower:8
- [Mate]: 100MMshockLower:8 ↔ 9002T445_Corrosion-Resistant Precision Compression Springs:8
- [Mate]: 100MMshockUpper:8 ↔ 9002T445_Corrosion-Resistant Precision Compression Springs:8
- [Mate]: 100MMshockUpper:8 ↔ springSpacerV1:5
- [Mate]: 100MMshockUpper:8 ↔ springSpacerV1:5
- [Mate]: swingarmBaseV4_mirror:4 ↔ 100MMshockUpper:8
- [Mate]: swingarmV2_mirrored:4 ↔ 100MMshockLower:8
- [Flush] (-2 mm): swingarmV2_mirrored:4 ↔ 100MMshockUpper:8
- [Mate]: swingarmBaseV4_mirror:4 ↔ 91290A270_Alloy Steel Socket Head Screw:4
- [Mate]: swingarmBaseV4_mirror:4 ↔ 91290A270_Alloy Steel Socket Head Screw:4
- [Mate]: 92981A203_Alloy Steel Shoulder Screws:16 ↔ 90237A130_High-Strength Steel Nylon-Insert Locknuts:15
- [Mate]: 6082rsBearing:55 ↔ 92981A203_Alloy Steel Shoulder Screws:16
- [Mate]: 6082rsBearing:55 ↔ 92981A203_Alloy Steel Shoulder Screws:16
- [Mate]: 92981A203_Alloy Steel Shoulder Screws:16 ↔ 90237A130_High-Strength Steel Nylon-Insert Locknuts:15
- [Mate]: swingarmV2_mirrored:4 ↔ 90237A130_High-Strength Steel Nylon-Insert Locknuts:15
- [Mate]: 92981A203_Alloy Steel Shoulder Screws:17 ↔ 90237A130_High-Strength Steel Nylon-Insert Locknuts:16
- [Mate]: 6082rsBearing:57 ↔ 92981A203_Alloy Steel Shoulder Screws:17
- [Mate]: 6082rsBearing:57 ↔ 92981A203_Alloy Steel Shoulder Screws:17
- [Mate]: 92981A203_Alloy Steel Shoulder Screws:17 ↔ 90237A130_High-Strength Steel Nylon-Insert Locknuts:16
- [Mate]: swingarmV2_mirrored:4 ↔ 90237A130_High-Strength Steel Nylon-Insert Locknuts:16
- Mate:427: trackBase:2 ↔ swingarmBaseV4_mirror:4
- Mate:428: trackBase:2 ↔ swingarmBaseV4_mirror:4
- Flush:27: swingarmBaseV2:4 ↔ swingarmBaseV4_mirror:4
- Flush:28: swingarmV2:4 ↔ swingarmV2_mirrored:4
- Flush:29: beltV2:1 ↔ beltV2:2
- Flush:30: beltV2:1 ↔ beltV2:2
- Flush:31: hoverboardPulleyAdapter:2 ↔ beltV2:2
- Mate:429 (254 mm): trackBase:1 ↔ trackBase:2
- Mate:430: trackBase:1 ↔ horizontalStrut:1
- Flush:32: trackBase:1 ↔ horizontalStrut:1
- Flush:33: horizontalStrut:1 ↔ horizontalStrut:2
- Mate:431: trackBase:1 ↔ horizontalStrut:2
- Mate:432: trackBase:2 ↔ 4844N132_T-Slotted Framing Structural Bracket:1
- Flush:34: horizontalStrut:1 ↔ 4844N132_T-Slotted Framing Structural Bracket:1
- Flush:35: trackBase:2 ↔ 4844N132_T-Slotted Framing Structural Bracket:1
- Mate:433: horizontalStrut:1 ↔ 4844N132_T-Slotted Framing Structural Bracket:4
- Flush:36: trackBase:1 ↔ 4844N132_T-Slotted Framing Structural Bracket:4
- Flush:37: horizontalStrut:1 ↔ 4844N132_T-Slotted Framing Structural Bracket:4
- Mate:434: horizontalStrut:2 ↔ 4844N132_T-Slotted Framing Structural Bracket:2
- Flush:38: trackBase:2 ↔ 4844N132_T-Slotted Framing Structural Bracket:2
- Flush:39: horizontalStrut:2 ↔ 4844N132_T-Slotted Framing Structural Bracket:2
- Mate:435: horizontalStrut:2 ↔ 4844N132_T-Slotted Framing Structural Bracket:3
- Flush:40: trackBase:1 ↔ 4844N132_T-Slotted Framing Structural Bracket:3
- Flush:41: horizontalStrut:2 ↔ 4844N132_T-Slotted Framing Structural Bracket:3
- Mate:436: trackBase:1 ↔ 4844N105_T-Slotted Framing Structural Bracket:1
- Mate:437: horizontalStrut:2 ↔ 4844N105_T-Slotted Framing Structural Bracket:1
- Flush:42 (2 mm): horizontalStrut:2 ↔ 4844N105_T-Slotted Framing Structural Bracket:1
- Mate:438: trackBase:2 ↔ 4844N105_T-Slotted Framing Structural Bracket:2
- Mate:439: horizontalStrut:2 ↔ 4844N105_T-Slotted Framing Structural Bracket:2
- Flush:43: 4844N105_T-Slotted Framing Structural Bracket:1 ↔ 4844N105_T-Slotted Framing Structural Bracket:2
- Mate:451: Motor driver ODRIVE V3.6:1 ↔ odriveAndBatteryMountV1:1
- Mate:452: Motor driver ODRIVE V3.6:1 ↔ odriveAndBatteryMountV1:1
- Mate:453: Motor driver ODRIVE V3.6:1 ↔ odriveAndBatteryMountV1:1
- Mate:454: 50W 2Ohm Power Resistor:1 ↔ odriveAndBatteryMountV1:1
- Mate:455: 50W 2Ohm Power Resistor:1 ↔ odriveAndBatteryMountV1:1
- Mate:456: 50W 2Ohm Power Resistor:1 ↔ odriveAndBatteryMountV1:1
- Mate:457: horizontalStrut:2 ↔ odriveAndBatteryMountV1:1
- Mate:458: horizontalStrut:2 ↔ odriveAndBatteryMountV1:1
- Mate:459: E-STOP:1 ↔ estopMountV1:1
- Mate:460: E-STOP:1 ↔ estopMountV1:1
- Mate:461: E-STOP:1 ↔ estopMountV1:1
- Mate:464: trackBase:1 ↔ LAPTOP:1
- Mate:466: horizontalStrut:1 ↔ estopMountV1:1
- Mate:467: horizontalStrut:2 ↔ estopMountV1:1
- Mate:468: hoverboardPulleyAdapter:1 ↔ hoverboardHubCap:1
- Mate:469: hoverboardPulleyAdapter:2 ↔ hoverboardHubCap:2
- Mate:470: hoverboardPulleyAdapter:2 ↔ hoverboardHubCap:2
- Mate:471: trackBase:2 ↔ laptopClampBase:1
- Flush:56: trackBase:2 ↔ laptopClampBase:1
- Mate:472: hoverboard_motor_assembly:2 ↔ hoverboardInnerHubCap:1
- Mate:473: hoverboard_motor_assembly:2 ↔ hoverboardInnerHubCap:1
- Mate:474: hoverboardInnerHubCap:1 ↔ hoverboardInnerHubCap:2
- Mate:475: hoverboardInnerHubCap:1 ↔ hoverboardInnerHubCap:3
- Flush:57: hoverboardInnerHubCap:1 ↔ hoverboardInnerHubCap:2
- Flush:58: hoverboardInnerHubCap:1 ↔ hoverboardInnerHubCap:3
- Mate:476: hoverboard_motor_assembly:2 ↔ hoverboardInnerHubCap:1
- Mate:477: hoverboard_motor_assembly:2 ↔ hoverboardInnerHubCap:3
- Mate:478: hoverboard_motor_assembly:2 ↔ hoverboardInnerHubCap:2
- [Mate]: hoverboardInnerHubCap:4 ↔ hoverboardInnerHubCap:5
- [Mate]: hoverboardInnerHubCap:4 ↔ hoverboardInnerHubCap:6
- [Flush]: hoverboardInnerHubCap:4 ↔ hoverboardInnerHubCap:5
- [Flush]: hoverboardInnerHubCap:4 ↔ hoverboardInnerHubCap:6
- Mate:481: hoverboard_motor_assembly:1 ↔ hoverboardInnerHubCap:4
- Mate:482: hoverboard_motor_assembly:1 ↔ hoverboardInnerHubCap:4
- Mate:483: hoverboard_motor_assembly:1 ↔ hoverboardInnerHubCap:4
- Mate:484: hoverboard_motor_assembly:1 ↔ hoverboardInnerHubCap:5
- Mate:485: hoverboard_motor_assembly:1 ↔ hoverboardInnerHubCap:6
- Mate:486: dellLatitudeBase:1 ↔ dellLatitudeScreen:1
- Mate:487: dellLatitudeBase:1 ↔ dellLatitudeScreen:1
- Flush:61: idlerBaseV1:1 ↔ idlerBaseV1:4
- Mate:488: laptopClampBase:1 ↔ laptopClampScrew:1
- Mate:489: laptopClampBase:1 ↔ laptopClampScrew:1
- Mate:490: trackBase:1 ↔ laptopClampBaseFlipped:1
- Mate:491: trackBase:1 ↔ laptopClampBaseFlipped:1
- Flush:62: laptopClampBase:1 ↔ laptopClampBaseFlipped:1
- Mate:492: laptopClampBaseFlipped:1 ↔ laptopClampScrew:2
- Mate:493: laptopClampBaseFlipped:1 ↔ laptopClampScrew:2
- Flush:63: horizontalStrut:4 ↔ horizontalStrut:5
- Flush:64: horizontalStrut:4 ↔ horizontalStrut:5
- Mate:494: trackBase:1 ↔ 12inStrut:1
- Flush:65: trackBase:1 ↔ 12inStrut:1
- Flush:66: trackBase:1 ↔ 12inStrut:1